# Autodesk Inventor assembly: OUTER TORSO
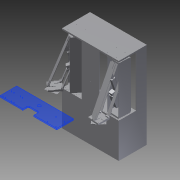
[picture p0: Inventor's stored thumbnail of the model, 180x180]
Saved by Autodesk Inventor 2011 (Build 150239000, 239)
## iProperties
Created: 2011-10-30
Part Number: OUTER TORSO
Document SubType Name: Assembly
Designer: Matthew
Author: Matthew
## Documents named in this file (6)
- C:\Users\Matthew\Documents\matthew_autocad\prlite\outer torso\OUTER TORSO.iam
- C:\Users\Matthew\Documents\matthew_autocad\prlite\outer torso\front.ipt
- C:\Users\Matthew\Documents\matthew_autocad\prlite\outer torso\holder.ipt
- C:\Users\Matthew\Documents\matthew_autocad\prlite\outer torso\side.ipt
- C:\Users\Matthew\Documents\matthew_autocad\prlite\outer torso\holdertop.ipt
- C:\Users\Matthew\Documents\matthew_autocad\prlite\arm perhaps\ARM PERHAPS use2.iam
## Components (6 placed, 5 different names)
1. front:1 — Mate:1, Mate:2, Flush:2, Flush:3, Mate:4, Flush:5, Flush:6, Flush:8, Flush:9, Mate:20
2. side:1 — Mate:1, Flush:3, Flush:8
3. side:2 — Mate:2, Flush:2, Flush:7, Flush:9, Flush:10
4. holder:1 — Mate:4, Flush:5, Flush:10, Mate:15, Mate:16
5. holdertop:1 — Flush:6, Flush:7, Mate:11, Mate:19, Mate:20
6. ARM PERHAPS use2:1 [sub-assembly] — Mate:11, Mate:15, Mate:16, Mate:19
## Relationships (16: Mate 8, Flush 8)
- Mate:1: front:1 ↔ side:1
- Mate:2: front:1 ↔ side:2
- Flush:2: front:1 ↔ side:2
- Flush:3: front:1 ↔ side:1
- Mate:4: front:1 ↔ holder:1
- Flush:5: front:1 ↔ holder:1
- Flush:6: front:1 ↔ holdertop:1
- Flush:7: side:2 ↔ holdertop:1
- Mate:11: holdertop:1 ↔ ARM PERHAPS use2:1
- Flush:8: front:1 ↔ side:1
- Flush:9: front:1 ↔ side:2
- Flush:10: side:2 ↔ holder:1
- Mate:15: holder:1 ↔ ARM PERHAPS use2:1
- Mate:16: holder:1 ↔ ARM PERHAPS use2:1
- Mate:19: holdertop:1 ↔ ARM PERHAPS use2:1
- Mate:20: front:1 ↔ holdertop:1
